# Autodesk Inventor assembly: Backplane
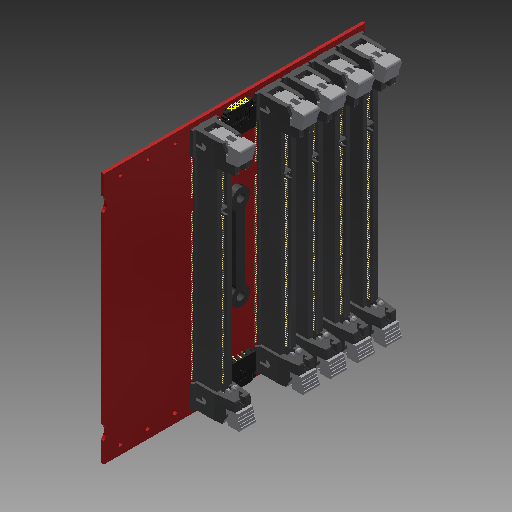
[picture p0: Inventor's stored thumbnail of the model, 512x512]
Saved by Autodesk Inventor 2018 (Build 220112000, 112)
## iProperties
Created: 2018-07-04
Part Number: Backplane
Document SubType Name: Assembly
Designer: Bradley
Mass: 32.9964 g
Surface Area: 520.338 cm^2
Volume: 30.2267 cm^3
Density: 1.09163 g/cm^3
Author: Bradley
## Documents named in this file (6)
- D:\Users\Bradley\Documents\CougsInSpace\CougSat1-Hardware\CougSat1-Backplane\CADModel\Native\Backplane.iam
- D:\Users\Bradley\Documents\CougsInSpace\CougSat1-Hardware\CougSat1-Backplane\CADModel\Native\Backplane_PCB.ipt
- D:\Users\Bradley\Documents\CougsInSpace\Resources\ComponentModels\Connectors\SODIMM-DDR.ipt
- D:\Users\Bradley\Documents\CougsInSpace\CougSat1-Hardware\CougSat1-Backplane\CADModel\Native\Backplane_Nut.ipt
- D:\Users\Bradley\Documents\CougsInSpace\Resources\ComponentModels\Connectors\PicoLock--J-4.ipt
- D:\Users\Bradley\Documents\CougsInSpace\Resources\ComponentModels\Connectors\PicoLock--P-4.ipt
## Components (11 placed, 5 different names)
1. Backplane_PCB:1 — Insert:1, Insert:2, Insert:3, Insert:4, Insert:5, Insert:6, Insert:13, Insert:14, Insert:15, Insert:16, Insert:17, Insert:18, Mate:1, Mate:6
2. Backplane_Nut:1 — Insert:17, Insert:18
3. PicoLock--J-4:1 — Mate:1, Mate:2, Mate:3, Flush:1, Flush:2, Flush:3
4. PicoLock--P-4:1 — Mate:2, Mate:3, Flush:1
5. PicoLock--J-4:2 — Mate:6, Mate:7, Mate:8
6. PicoLock--P-4:2
7. SODIMM-DDR:1 — Insert:1, Insert:2
8. SODIMM-DDR:2 — Insert:3, Insert:16
9. SODIMM-DDR:3 — Insert:4, Insert:15
10. SODIMM-DDR:4 — Insert:5, Insert:14
11. SODIMM-DDR:5 — Insert:6, Insert:13
## Relationships (24: Insert 12, Mate 8, Flush 4)
- Insert:1: Backplane_PCB:1 ↔ SODIMM-DDR:1
- Insert:2: Backplane_PCB:1 ↔ SODIMM-DDR:1
- Insert:3: Backplane_PCB:1 ↔ SODIMM-DDR:2
- Insert:4: Backplane_PCB:1 ↔ SODIMM-DDR:3
- Insert:5: Backplane_PCB:1 ↔ SODIMM-DDR:4
- Insert:6: Backplane_PCB:1 ↔ SODIMM-DDR:5
- Insert:13: Backplane_PCB:1 ↔ SODIMM-DDR:5
- Insert:14: Backplane_PCB:1 ↔ SODIMM-DDR:4
- Insert:15: Backplane_PCB:1 ↔ SODIMM-DDR:3
- Insert:16: Backplane_PCB:1 ↔ SODIMM-DDR:2
- Insert:17: Backplane_PCB:1 ↔ Backplane_Nut:1
- Insert:18: Backplane_PCB:1 ↔ Backplane_Nut:1
- Mate:1: Backplane_PCB:1 ↔ PicoLock--J-4:1
- Mate:2 (0.04 mm): PicoLock--J-4:1 ↔ PicoLock--P-4:1
- Mate:3: PicoLock--J-4:1 ↔ PicoLock--P-4:1
- Flush:1: PicoLock--J-4:1 ↔ PicoLock--P-4:1
- Flush:2 (32 mm): PicoLock--J-4:1
- Flush:3: PicoLock--J-4:1
- [Mate] (0.04 mm): PicoLock--J-4:2 ↔ PicoLock--P-4:2
- [Mate]: PicoLock--J-4:2 ↔ PicoLock--P-4:2
- [Flush]: PicoLock--J-4:2 ↔ PicoLock--P-4:2
- Mate:6: Backplane_PCB:1 ↔ PicoLock--J-4:2
- Mate:7 (32 mm): PicoLock--J-4:2
- Mate:8: PicoLock--J-4:2
## Named parameters: d24_d19 = 0.04 mm, d25_d20 = 0 mm, d26_d21 = 0 mm
